# Autodesk Inventor assembly: MONTAGEM_COMPLETA
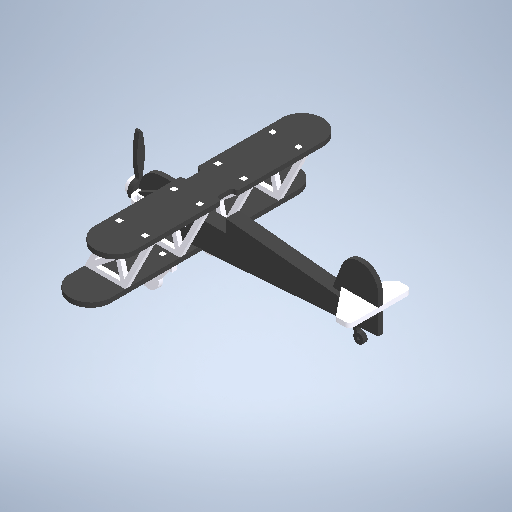
[picture p0: Inventor's stored thumbnail of the model, 512x512]
Saved by Autodesk Inventor 2025.1 (Build 291241000, 241)
## iProperties
Created: 2024-10-26
Part Number: MONTAGEM_COMPLETA
Document SubType Name: Assembly
Designer: ambrosildo
Author: ambrosildo
## Documents named in this file (10)
- C:\my-docs\Inventor\aeroscorpion\MONTAGEM_COMPLETA.iam
- C:\my-docs\Inventor\aeroscorpion\CORPO.ipt
- C:\my-docs\Inventor\aeroscorpion\ASA_INFERIOR.ipt
- C:\my-docs\Inventor\aeroscorpion\RODAl.ipt
- C:\my-docs\Inventor\aeroscorpion\MOTOR.ipt
- C:\my-docs\Inventor\aeroscorpion\LEME.ipt
- C:\my-docs\Inventor\aeroscorpion\ENTRE_ASA.ipt
- C:\my-docs\Inventor\aeroscorpion\ASA_SUPERIOR.ipt
- C:\my-docs\Inventor\aeroscorpion\HELICE.ipt
- C:\my-docs\Inventor\aeroscorpion\TRAVA_HELICE.ipt
## Components (13 placed, 9 different names)
1. CORPO:1 — Rígida:1, Rígida:4, Rígida:5
2. ASA_INFERIOR:1 — Rígida:1, Rígida:2, Rígida:3, Rígida:6, Rígida:7, Rígida:8, Rígida:9
3. RODAl:1 — Rígida:3
4. RODAl:2 — Rígida:2
5. MOTOR:1 — Rígida:4, Rígida:11, Rígida:12
6. LEME:1 — Rígida:5
7. ENTRE_ASA:1 — Rígida:9
8. ENTRE_ASA:2 — Rígida:8
9. ENTRE_ASA:3 — Rígida:7
10. ENTRE_ASA:4 — Rígida:6, Rígida:10
11. ASA_SUPERIOR:1 — Rígida:10
12. HELICE:1 — Rígida:11
13. TRAVA_HELICE:1 — Rígida:12
## Relationships (12: WeldJoint 12)
- Rígida:1 [WeldJoint]: CORPO:1 ↔ ASA_INFERIOR:1
- Rígida:2 [WeldJoint]: ASA_INFERIOR:1 ↔ RODAl:2
- Rígida:3 [WeldJoint]: ASA_INFERIOR:1 ↔ RODAl:1
- Rígida:4 [WeldJoint]: CORPO:1 ↔ MOTOR:1
- Rígida:5 [WeldJoint]: CORPO:1 ↔ LEME:1
- Rígida:6 [WeldJoint]: ASA_INFERIOR:1 ↔ ENTRE_ASA:4
- Rígida:7 [WeldJoint]: ASA_INFERIOR:1 ↔ ENTRE_ASA:3
- Rígida:8 [WeldJoint]: ASA_INFERIOR:1 ↔ ENTRE_ASA:2
- Rígida:9 [WeldJoint]: ASA_INFERIOR:1 ↔ ENTRE_ASA:1
- Rígida:10 [WeldJoint]: ENTRE_ASA:4 ↔ ASA_SUPERIOR:1
- Rígida:11 [WeldJoint] (-6.25 mm): MOTOR:1 ↔ HELICE:1
- Rígida:12 [WeldJoint]: MOTOR:1 ↔ TRAVA_HELICE:1
## Named parameters: Finish10_Area = 37.5057, Finish11_Area = 17.3346, Finish12_Area = 1.44, Finish13_Area = 0.12, Finish14_Area = 0.6, Finish15_Area = 19.2012, Finish16_Area = 19.1773, Finish17_Area = 19.2161, Finish18_Area = 19.2161, Finish19_Area = 3.06301, Finish1_Area = 7.43917, Finish20_Area = 13.3823, Finish21_Area = 7.39854, Finish2_Area = 1.3944, Finish3_Area = 94.5876, Finish4_Area = 8.84003, Finish5_Area = 0.09, Finish6_Area = 101.582, Finish7_Area = 11.6831, Finish8_Area = 16.4977, Finish9_Area = 37.1607
note: some values were not read from the file. Shown as the stored number, unit unknown: "Finish10_Area", "Finish11_Area", "Finish12_Area", "Finish13_Area", "Finish14_Area", "Finish15_Area", "Finish16_Area", "Finish17_Area", "Finish18_Area", "Finish19_Area", "Finish1_Area", "Finish20_Area", "Finish21_Area", "Finish2_Area", "Finish3_Area", "Finish4_Area", "Finish5_Area", "Finish6_Area", "Finish7_Area", "Finish8_Area", "Finish9_Area".
